# Autodesk Inventor assembly: standoff_brace_triangle_mirrored
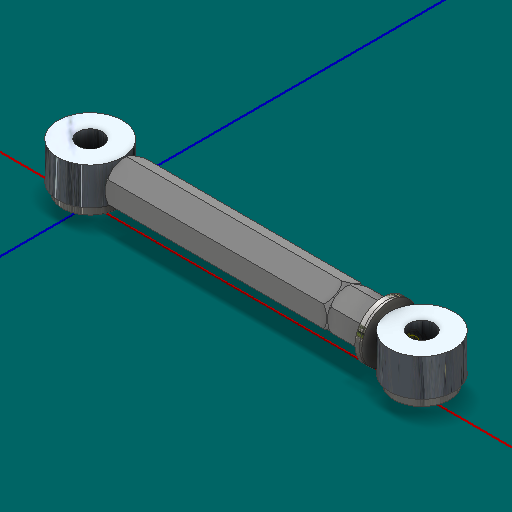
[picture p0: Inventor's stored thumbnail of the model, 512x512]
Saved by Autodesk Inventor 2025 (Build 290162000, 162)
## iProperties
Created: 2024-08-17
Part Number: standoff_brace_triangle_mirrored
Document SubType Name: Assembly
Designer: averey
Author: averey
## Documents named in this file (9)
- C:\Users\avere\vex_robotics_high_stakes\hardware\cad\ATLAS\chassis\structure\rail_mirrored\standoff_brace_triangle_mirrored.iam
- C:\Users\avere\vex_robotics_high_stakes\hardware\cad\ATLAS\chassis\structure\rail_mirrored\Shaft Collar No Screw_mirrored.ipt
- C:\Users\avere\vex_robotics_high_stakes\hardware\cad\VEX-CAD-Inventor\Structure\Standoff\Standoff .25.ipt
- C:\Users\avere\vex_robotics_high_stakes\hardware\cad\VEX-CAD-Inventor\Structure\Standoff.ipt
- C:\Users\avere\vex_robotics_high_stakes\hardware\cad\VEX-CAD-Inventor\Structure\Standoff\Standoff 1.50.ipt
- C:\Users\avere\vex_robotics_high_stakes\hardware\cad\VEX-CAD-Inventor\Motion\Spacers\Washer Steel\SWasher .375 OD x .015625.ipt
- C:\Users\avere\vex_robotics_high_stakes\hardware\cad\VEX-CAD-Inventor\Motion\Spacers\Washer Steel.ipt
- C:\Users\avere\vex_robotics_high_stakes\hardware\cad\VEX-CAD-Inventor\Motion\Spacers\Washer Steel\SWasher .375 OD x .031250.ipt
- C:\Users\avere\vex_robotics_high_stakes\hardware\cad\VEX-CAD-Inventor\Motion\Spacers\Washer Steel\SWasher .375 OD x .062500.ipt
## Components (8 placed, 6 different names)
1. Shaft Collar No Screw_mirrored:1 — Angle:2, Mate:2, Insert:5, Mate:1, Insert:7
2. Shaft Collar No Screw_mirrored:2 — Angle:3, Insert:5, Mate:1, Insert:4, Insert:6
3. Standoff .25:1 — Insert:1, Insert:3
4. Standoff 1.50:2 — Angle:1, Insert:1
5. SWasher .375 OD x .015625:1 — Insert:4, Insert:2
6. SWasher .375 OD x .031250:2 — Insert:3, Insert:2
7. SWasher .375 OD x .062500:3 — Insert:6
8. SWasher .375 OD x .062500:4 — Insert:7
## Relationships (12: Insert 7, Angle 3, Mate 2)
- Angle:2 (0 deg): Shaft Collar No Screw_mirrored:1
- Mate:2: Shaft Collar No Screw_mirrored:1
- Angle:3 (0 deg): Shaft Collar No Screw_mirrored:2
- Insert:5 (45.7961 mm): Shaft Collar No Screw_mirrored:1 ↔ Shaft Collar No Screw_mirrored:2
- Mate:1: Shaft Collar No Screw_mirrored:1 ↔ Shaft Collar No Screw_mirrored:2
- Angle:1 (0 deg): Standoff 1.50:2
- Insert:1: Standoff .25:1 ↔ Standoff 1.50:2
- Insert:4: Shaft Collar No Screw_mirrored:2 ↔ SWasher .375 OD x .015625:1
- Insert:3: Standoff .25:1 ↔ SWasher .375 OD x .031250:2
- Insert:2: SWasher .375 OD x .015625:1 ↔ SWasher .375 OD x .031250:2
- Insert:6: Shaft Collar No Screw_mirrored:2 ↔ SWasher .375 OD x .062500:3
- Insert:7: Shaft Collar No Screw_mirrored:1 ↔ SWasher .375 OD x .062500:4
